# Autodesk Inventor assembly: Arm_MiniLink_Shim_i_9
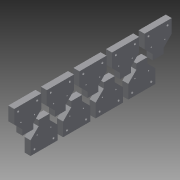
[picture p0: Inventor's stored thumbnail of the model, 180x180]
Saved by Autodesk Inventor 2013 (Build 170138000, 138)
## iProperties
Created: 2014-05-17
Part Number: Arm_MiniLink_Shim_i_9
Document SubType Name: Assembly
Designer: andou
Author: andou
## Documents named in this file (3)
- C:\Users\andou\Documents\Inventor\RoboticsProject\project_4\Robot\Arm\Arm_MiniLink_Shim_i_9.iam
- C:\Users\andou\Documents\Inventor\RoboticsProject\project_4\Robot\Arm\Arm_MiniLink_Shim_i_5.iam
- C:\Users\andou\Documents\Inventor\RoboticsProject\project_4\Robot\Arm\Arm_MiniLink_Shim_i_4.iam
## Components (2 placed, 2 different names)
1. Arm_MiniLink_Shim_i_5:1 [sub-assembly] — メイト:1, フラッシュ:1, メイト:2
2. Arm_MiniLink_Shim_i_4:1 [sub-assembly] — メイト:1, フラッシュ:1, メイト:2
## Relationships (3: Mate 2, Flush 1)
- メイト:1 [Mate] (-10 mm): Arm_MiniLink_Shim_i_5:1 ↔ Arm_MiniLink_Shim_i_4:1
- フラッシュ:1 [Flush]: Arm_MiniLink_Shim_i_5:1 ↔ Arm_MiniLink_Shim_i_4:1
- メイト:2 [Mate] (10 mm): Arm_MiniLink_Shim_i_5:1 ↔ Arm_MiniLink_Shim_i_4:1
